# Autodesk Inventor assembly: MK2_TopFrame
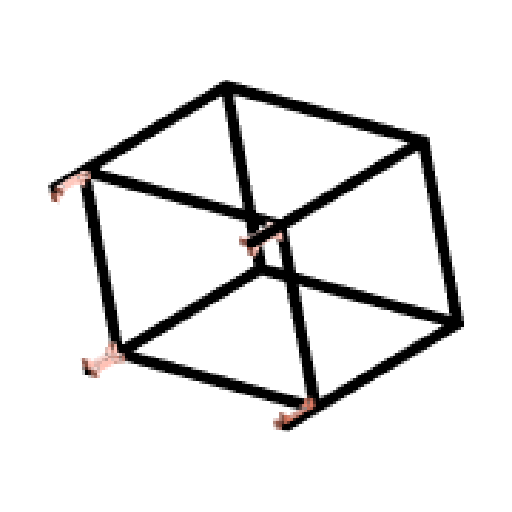
[picture p0: Inventor's stored thumbnail of the model, 512x512]
Saved by Autodesk Inventor 2023.2 (Build 272271000, 271)
## iProperties
Created: 2020-05-24
Part Number: MK2_TopFrame
Document SubType Name: Assembly
Designer: Remo
Description: H-Bot Printer Subassembly / Bottom Frame
Author: Remo
Revision Number: 2
## Documents named in this file (8)
- C:\Users\remop\OneDrive\Documents\Inventor\3D Printers\LuEVO\Mk5_FullKinematic\Mk5_TopFrame.iam
- C:\Users\remop\OneDrive\Documents\Inventor\3D Printers\LuEVO\Mk5_FullKinematic\Makerbeam\Beam_450mm.ipt
- C:\Users\remop\OneDrive\Documents\Inventor\3D Printers\LuEVO\Mk5_FullKinematic\Makerbeam\Beam_360mm.ipt
- C:\Users\remop\OneDrive\Documents\Inventor\3D Printers\LuEVO\Mk5_FullKinematic\Makerbeam\Beam_CornerCube.ipt
- C:\Users\remop\OneDrive\Documents\Inventor\3D Printers\LuEVO\Mk5_FullKinematic\Makerbeam\Beam_500mm.ipt
- C:\Users\remop\OneDrive\Documents\Inventor\3D Printers\LuEVO\Mk5_FullKinematic\Makerbeam\Beam_CornerTri.ipt
- C:\Users\remop\OneDrive\Documents\Inventor\3D Printers\LuEVO\Mk5_FullKinematic\Frame Brace Mount.ipt
- C:\Users\remop\OneDrive\Documents\Inventor\Content Center Files\R2023\en-US\AS 1420\AS 1420 - 1973 - M3 x 6.ipt
## Components (57 placed, 7 different names)
1. Frame Brace Mount:1 — Mate:35, Flush:33, Flush:34, Mate:36, Insert:27, Insert:28, Insert:29, Insert:31
2. Frame Brace Mount:2 — Mate:37, Mate:38, Flush:35, Insert:1, Insert:2, Insert:3, Insert:4
3. Frame Brace Mount:3 — Mate:39, Flush:36, Flush:37, Mate:40, Insert:19, Insert:20, Insert:21, Insert:23
4. Frame Brace Mount:4 — Mate:41, Mate:42, Flush:38, Insert:11, Insert:12, Mate:50, Mate:51, Insert:14
5. Beam_500mm:4 — Mate:43, Flush:39, Flush:40, Flush:42, Flush:43, Mate:44
6. Frame Brace Mount:5 — Flush:42, Flush:43, Mate:44, Mate:47, Flush:48, Flush:49, Insert:16, Insert:17, Insert:18, Insert:22
7. Frame Brace Mount:6 — Mate:43, Flush:39, Flush:40, Insert:24, Insert:25, Insert:26, Insert:30
8. Beam_500mm:5 — Flush:51
9. Frame Brace Mount:7 — Mate:48, Insert:5, Insert:6, Insert:7, Insert:8
10. Frame Brace Mount:8 — Flush:52, Mate:49, Insert:9, Insert:10, Insert:13, Insert:15
11. AS 1420 - Metric M3 x 6:1 — Insert:1
12. AS 1420 - Metric M3 x 6:2 — Insert:2
13. AS 1420 - Metric M3 x 6:3 — Insert:3
14. AS 1420 - Metric M3 x 6:4 — Insert:4
15. AS 1420 - Metric M3 x 6:5 — Insert:5
16. AS 1420 - Metric M3 x 6:6 — Insert:6
17. AS 1420 - Metric M3 x 6:7 — Insert:7
18. AS 1420 - Metric M3 x 6:8 — Insert:8
19. AS 1420 - Metric M3 x 6:9 — Insert:9
20. AS 1420 - Metric M3 x 6:10 — Insert:10
21. AS 1420 - Metric M3 x 6:11 — Insert:11
22. AS 1420 - Metric M3 x 6:12 — Insert:12
23. AS 1420 - Metric M3 x 6:13 — Mate:50, Mate:51
24. AS 1420 - Metric M3 x 6:14 — Insert:13
25. AS 1420 - Metric M3 x 6:15 — Insert:14
26. AS 1420 - Metric M3 x 6:16 — Insert:15
27. AS 1420 - Metric M3 x 6:17 — Insert:16
28. AS 1420 - Metric M3 x 6:18 — Insert:17
29. AS 1420 - Metric M3 x 6:19 — Insert:18
30. AS 1420 - Metric M3 x 6:20 — Insert:19
31. AS 1420 - Metric M3 x 6:21 — Insert:20
32. AS 1420 - Metric M3 x 6:22 — Insert:21
33. AS 1420 - Metric M3 x 6:23 — Insert:22
34. AS 1420 - Metric M3 x 6:24 — Insert:23
35. AS 1420 - Metric M3 x 6:25 — Insert:24
36. AS 1420 - Metric M3 x 6:26 — Insert:25
37. AS 1420 - Metric M3 x 6:27 — Insert:26
38. AS 1420 - Metric M3 x 6:28 — Insert:27
39. AS 1420 - Metric M3 x 6:29 — Insert:28
40. AS 1420 - Metric M3 x 6:30 — Insert:29
41. AS 1420 - Metric M3 x 6:31 — Insert:30
42. AS 1420 - Metric M3 x 6:32 — Insert:31
43. Beam_CornerCube:4 — Rigid:4, Rigid:6, Rigid:10
44. Beam_CornerCube:3 — Rigid:3, Rigid:5, Rigid:11
45. Beam_CornerCube:1 — Rigid:8, Rigid:1, Rigid:12
46. Beam_CornerCube:2 — Rigid:2, Rigid:7
47. Beam_500mm:2 — Rigid:11, Rigid:12
48. Beam_360mm:1 — Rigid:5, Rigid:6
49. Beam_500mm:1 — Rigid:10
50. Beam_360mm:2 — Rigid:7, Rigid:8
51. Beam_450mm:2 — Rigid:2, Mate:4, Flush:1, Mate:41, Flush:51, Flush:52, Mate:49
52. Beam_450mm:1 — Rigid:1, Flush:36, Flush:37, Mate:40, Mate:47, Flush:48, Flush:49
53. Beam_450mm:4 — Rigid:4, Mate:2, Flush:2, Mate:37, Flush:35, Mate:48
54. Beam_450mm:3 — Rigid:3, Mate:25, Flush:20, Flush:21, Mate:35, Flush:33, Flush:34
55. Beam_CornerTri:9 — Mate:25, Flush:20, Flush:21
56. Beam_360mm:3 — Mate:2, Flush:2, Mate:36, Mate:38
57. Beam_360mm:4 — Mate:4, Flush:1, Mate:39, Mate:42, Flush:38
## Relationships (83: Insert 31, Flush 21, Mate 20, WeldJoint 11)
- Rigid:2 [WeldJoint]: Beam_CornerCube:2 ↔ Beam_450mm:2
- Rigid:3 [WeldJoint]: Beam_CornerCube:3 ↔ Beam_450mm:3
- Rigid:4 [WeldJoint]: Beam_CornerCube:4 ↔ Beam_450mm:4
- Rigid:5 [WeldJoint]: Beam_CornerCube:3 ↔ Beam_360mm:1
- Rigid:6 [WeldJoint]: Beam_CornerCube:4 ↔ Beam_360mm:1
- Rigid:7 [WeldJoint]: Beam_CornerCube:2 ↔ Beam_360mm:2
- Rigid:8 [WeldJoint]: Beam_CornerCube:1 ↔ Beam_360mm:2
- Rigid:1 [WeldJoint]: Beam_CornerCube:1 ↔ Beam_450mm:1
- Rigid:10 [WeldJoint]: Beam_CornerCube:4 ↔ Beam_500mm:1
- Rigid:11 [WeldJoint]: Beam_CornerCube:3 ↔ Beam_500mm:2
- Rigid:12 [WeldJoint]: Beam_CornerCube:1 ↔ Beam_500mm:2
- Mate:2: Beam_450mm:4 ↔ Beam_360mm:3
- Mate:4: Beam_450mm:2 ↔ Beam_360mm:4
- Flush:1: Beam_450mm:2 ↔ Beam_360mm:4
- Flush:2: Beam_450mm:4 ↔ Beam_360mm:3
- Mate:25: Beam_450mm:3 ↔ Beam_CornerTri:9
- Flush:20: Beam_450mm:3 ↔ Beam_CornerTri:9
- Flush:21: Beam_450mm:3 ↔ Beam_CornerTri:9
- Mate:35: Frame Brace Mount:1 ↔ Beam_450mm:3
- Flush:33: Frame Brace Mount:1 ↔ Beam_450mm:3
- Flush:34: Frame Brace Mount:1 ↔ Beam_450mm:3
- Mate:36: Frame Brace Mount:1 ↔ Beam_360mm:3
- Mate:37: Frame Brace Mount:2 ↔ Beam_450mm:4
- Mate:38: Frame Brace Mount:2 ↔ Beam_360mm:3
- Flush:35: Frame Brace Mount:2 ↔ Beam_450mm:4
- Mate:39: Frame Brace Mount:3 ↔ Beam_360mm:4
- Flush:36: Frame Brace Mount:3 ↔ Beam_450mm:1
- Flush:37: Frame Brace Mount:3 ↔ Beam_450mm:1
- Mate:40: Frame Brace Mount:3 ↔ Beam_450mm:1
- Mate:41: Frame Brace Mount:4 ↔ Beam_450mm:2
- Mate:42: Frame Brace Mount:4 ↔ Beam_360mm:4
- Flush:38: Frame Brace Mount:4 ↔ Beam_360mm:4
- Mate:43: Beam_500mm:4 ↔ Frame Brace Mount:6
- Flush:39: Beam_500mm:4 ↔ Frame Brace Mount:6
- Flush:40: Beam_500mm:4 ↔ Frame Brace Mount:6
- Flush:42: Beam_500mm:4 ↔ Frame Brace Mount:5
- Flush:43: Beam_500mm:4 ↔ Frame Brace Mount:5
- Mate:44: Beam_500mm:4 ↔ Frame Brace Mount:5
- [Mate]: Beam_500mm:5 ↔ Frame Brace Mount:8
- [Flush]: Beam_500mm:5 ↔ Frame Brace Mount:8
- [Flush]: Beam_500mm:5 ↔ Frame Brace Mount:7
- [Flush]: Beam_500mm:5 ↔ Frame Brace Mount:7
- [Mate]: Beam_500mm:5 ↔ Frame Brace Mount:7
- Mate:47: Frame Brace Mount:5 ↔ Beam_450mm:1
- Flush:48: Frame Brace Mount:5 ↔ Beam_450mm:1
- Flush:49: Frame Brace Mount:5 ↔ Beam_450mm:1
- Flush:51: Beam_500mm:5 ↔ Beam_450mm:2
- Flush:52: Frame Brace Mount:8 ↔ Beam_450mm:2
- Mate:48: Frame Brace Mount:7 ↔ Beam_450mm:4
- Mate:49: Frame Brace Mount:8 ↔ Beam_450mm:2
- Insert:1: Frame Brace Mount:2 ↔ AS 1420 - Metric M3 x 6:1
- Insert:2: Frame Brace Mount:2 ↔ AS 1420 - Metric M3 x 6:2
- Insert:3: Frame Brace Mount:2 ↔ AS 1420 - Metric M3 x 6:3
- Insert:4: Frame Brace Mount:2 ↔ AS 1420 - Metric M3 x 6:4
- Insert:5: Frame Brace Mount:7 ↔ AS 1420 - Metric M3 x 6:5
- Insert:6: Frame Brace Mount:7 ↔ AS 1420 - Metric M3 x 6:6
- Insert:7: Frame Brace Mount:7 ↔ AS 1420 - Metric M3 x 6:7
- Insert:8: Frame Brace Mount:7 ↔ AS 1420 - Metric M3 x 6:8
- Insert:9: Frame Brace Mount:8 ↔ AS 1420 - Metric M3 x 6:9
- Insert:10: Frame Brace Mount:8 ↔ AS 1420 - Metric M3 x 6:10
- Insert:11: Frame Brace Mount:4 ↔ AS 1420 - Metric M3 x 6:11
- Insert:12: Frame Brace Mount:4 ↔ AS 1420 - Metric M3 x 6:12
- Mate:50: Frame Brace Mount:4 ↔ AS 1420 - Metric M3 x 6:13
- Mate:51: Frame Brace Mount:4 ↔ AS 1420 - Metric M3 x 6:13
- Insert:13: Frame Brace Mount:8 ↔ AS 1420 - Metric M3 x 6:14
- Insert:14: Frame Brace Mount:4 ↔ AS 1420 - Metric M3 x 6:15
- Insert:15: Frame Brace Mount:8 ↔ AS 1420 - Metric M3 x 6:16
- Insert:16: Frame Brace Mount:5 ↔ AS 1420 - Metric M3 x 6:17
- Insert:17: Frame Brace Mount:5 ↔ AS 1420 - Metric M3 x 6:18
- Insert:18: Frame Brace Mount:5 ↔ AS 1420 - Metric M3 x 6:19
- Insert:19: Frame Brace Mount:3 ↔ AS 1420 - Metric M3 x 6:20
- Insert:20: Frame Brace Mount:3 ↔ AS 1420 - Metric M3 x 6:21
- Insert:21: Frame Brace Mount:3 ↔ AS 1420 - Metric M3 x 6:22
- Insert:22: Frame Brace Mount:5 ↔ AS 1420 - Metric M3 x 6:23
- Insert:23: Frame Brace Mount:3 ↔ AS 1420 - Metric M3 x 6:24
- Insert:24: Frame Brace Mount:6 ↔ AS 1420 - Metric M3 x 6:25
- Insert:25: Frame Brace Mount:6 ↔ AS 1420 - Metric M3 x 6:26
- Insert:26: Frame Brace Mount:6 ↔ AS 1420 - Metric M3 x 6:27
- Insert:27: Frame Brace Mount:1 ↔ AS 1420 - Metric M3 x 6:28
- Insert:28: Frame Brace Mount:1 ↔ AS 1420 - Metric M3 x 6:29
- Insert:29: Frame Brace Mount:1 ↔ AS 1420 - Metric M3 x 6:30
- Insert:30: Frame Brace Mount:6 ↔ AS 1420 - Metric M3 x 6:31
- Insert:31: Frame Brace Mount:1 ↔ AS 1420 - Metric M3 x 6:32
## Named parameters: d213_d206 = 0 mm, d215_d208 = 0 mm, d216_d210 = 0 mm, d217_d211 = 0 mm, d218_d212 = 0 mm
